# Autodesk Inventor assembly: drivetrain.asm
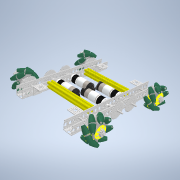
[picture p0: Inventor's stored thumbnail of the model, 180x180]
Saved by Autodesk Inventor 2020 (Build 240168000, 168)
## iProperties
Created: 2019-09-15
Part Number: drivetrain.asm
Document SubType Name: Assembly
Designer: tdmp4
Author: tdmp4
## Documents named in this file (23)
- C:\Users\tdmp4\OneDrive\Documents\GitHub\CAD-2020\Drivetrain\drivetrain.asm.iam
- C:\Users\tdmp4\OneDrive\Documents\GitHub\CAD-2020\ServoCity\585462_cut_17-5.ipt
- C:\Users\tdmp4\OneDrive\Documents\GitHub\CAD-2020\ServoCity\585424.ipt
- C:\Users\tdmp4\OneDrive\Documents\GitHub\CAD-2020\Drivetrain\4_Mecanum_Wheel_276-1447.ipt
- C:\Users\tdmp4\OneDrive\Documents\GitHub\CAD-2020\Drivetrain\GoodAdap.ipt
- C:\Users\tdmp4\OneDrive\Documents\GitHub\CAD-2020\Drivetrain\MirrorGoodAdap.ipt
- C:\Users\tdmp4\OneDrive\Documents\GitHub\CAD-2020\ServoCity\535198.ipt
- C:\Users\tdmp4\OneDrive\Documents\GitHub\CAD-2020\ServoCity\634080.ipt
- C:\Users\tdmp4\OneDrive\Documents\GitHub\CAD-2020\ServoCity\545619 assembly_MIR.ipt
- C:\Users\tdmp4\OneDrive\Documents\GitHub\CAD-2020\ServoCity\615114.ipt
- C:\Users\tdmp4\OneDrive\Documents\GitHub\CAD-2020\ServoCity\555128 assembly.ipt
- C:\Users\tdmp4\OneDrive\Documents\GitHub\CAD-2020\AndyMark\am-3637 NeveRest Orbital 20 Gearmotor REV2.ipt
- C:\Users\tdmp4\OneDrive\Documents\GitHub\CAD-2020\ServoCity\625051 assembly.ipt
- C:\Users\tdmp4\OneDrive\Documents\GitHub\CAD-2020\ServoCity\585462_cut_17-5_MIR.ipt
- C:\Users\tdmp4\OneDrive\Documents\GitHub\CAD-2020\ServoCity\585424_MIR.ipt
- C:\Users\tdmp4\OneDrive\Documents\GitHub\CAD-2020\Drivetrain\4_Mecanum_Wheel_276-1447_MIR.ipt
- C:\Users\tdmp4\OneDrive\Documents\GitHub\CAD-2020\Drivetrain\GoodAdap_MIR.ipt
- C:\Users\tdmp4\OneDrive\Documents\GitHub\CAD-2020\Drivetrain\MirrorGoodAdap_MIR.ipt
- C:\Users\tdmp4\OneDrive\Documents\GitHub\CAD-2020\ServoCity\535198_MIR.ipt
- C:\Users\tdmp4\OneDrive\Documents\GitHub\CAD-2020\ServoCity\634080_MIR.ipt
- C:\Users\tdmp4\OneDrive\Documents\GitHub\CAD-2020\ServoCity\615114_MIR.ipt
- C:\Users\tdmp4\OneDrive\Documents\GitHub\CAD-2020\Drivetrain\1010-Yellow-8_5-CL.ipt
- C:\Users\tdmp4\OneDrive\Documents\GitHub\CAD-2020\ServoCity\634068.ipt
## Components (72 placed, 22 different names)
1. 585462_cut_17-5:1 — Mate:1, Mate:2, Mate:3, Mate:17, Mate:18, Mate:33, Mate:34, Mate:35, Mate:38, Mate:39, Mate:57, Mate:58, Mate:59, Flush:4, Mate:62, Mate:63, Mate:64, Mate:68, Mate:70, Mate:71, Mate:72, Mate:73, Mate:74, Mate:154, Mate:156
2. 585424:1 — Mate:1, Mate:2, Mate:3, Mate:15, Mate:16
3. 4_Mecanum_Wheel_276-1447:1 — Mate:11, Mate:12, Mate:13, Mate:14
4. 4_Mecanum_Wheel_276-1447:2 — Mate:40, Mate:41, Mate:42, Mate:43
5. GoodAdap:1 — Mate:11, Mate:12, Mate:23, Mate:24, Mate:25
6. MirrorGoodAdap:1 — Mate:13, Mate:14, Mate:26, Mate:27, Mate:28, Mate:31
7. 535198:1 — Mate:15, Mate:16, Flush:2
8. 535198:2 — Mate:17, Mate:18, Mate:19
9. 634080:1 — Flush:2, Mate:19, Mate:32
10. 545619 assembly_MIR:1 — Mate:29, Mate:30, Mate:31, Mate:32, Mate:33
11. 545619 assembly_MIR:2 — Mate:23, Mate:24, Mate:25
12. 615114:1 — Mate:26, Mate:27, Mate:28, Mate:29, Mate:30
13. 585424:2 — Mate:34, Mate:35, Mate:36, Mate:37, Flush:4
14. 535198:3 — Mate:36, Mate:37, Mate:54, Flush:3
15. 535198:4 — Mate:38, Mate:39, Mate:56
16. MirrorGoodAdap:2 — Mate:40, Mate:41, Mate:44, Mate:45, Mate:46
17. GoodAdap:2 — Mate:42, Mate:43, Mate:51, Mate:52, Mate:53
18. 615114:2 — Mate:44, Mate:45, Mate:46, Mate:47, Mate:48, Mate:49, Mate:50
19. 545619 assembly_MIR:3 — Mate:47, Mate:48, Mate:49, Mate:50, Mate:55, Mate:56
20. 545619 assembly_MIR:4 — Mate:51, Mate:52, Mate:53
21. 634080:2 — Mate:54, Flush:3, Mate:55
22. 555128 assembly:1 — Mate:57, Mate:58, Mate:59, Mate:60, Mate:61
23. 555128 assembly:2 — Mate:62, Mate:63, Mate:64, Mate:65, Mate:66
24. am-3637 NeveRest Orbital 20 Gearmotor REV2:1 — Mate:60, Mate:61, Mate:69, Mate:163
25. am-3637 NeveRest Orbital 20 Gearmotor REV2:2 — Mate:65, Mate:66, Mate:67, Mate:161
26. 625051 assembly:1 — Mate:67, Mate:68
27. 625051 assembly:2 — Mate:69, Mate:70
28. 535198:5 — Mate:71, Mate:72, Mate:162, Mate:178
29. 535198:6 — Mate:73, Mate:74, Mate:160, Mate:176
30. 585462_cut_17-5_MIR:1 — Mate:75, Mate:76, Mate:77, Mate:84, Mate:85, Mate:87, Flush:6, Mate:98, Mate:99, Mate:102, Mate:103, Mate:144, Mate:145, Mate:146, Mate:147, Mate:148, Mate:149, Flush:11, Mate:164, Mate:165, Mate:166, Mate:167, Mate:175
31. 585424_MIR:1 — Mate:75, Mate:76, Mate:77, Mate:82, Mate:83
32. 4_Mecanum_Wheel_276-1447_MIR:1 — Mate:78, Mate:79, Mate:80, Mate:81
33. 4_Mecanum_Wheel_276-1447_MIR:2 — Mate:104, Mate:105, Mate:106, Mate:107
34. GoodAdap_MIR:1 — Mate:78, Mate:79, Mate:90, Mate:91, Mate:92
35. MirrorGoodAdap_MIR:1 — Mate:80, Mate:81, Mate:89, Mate:95, Mate:96, Mate:97
36. 535198_MIR:1 — Mate:82, Mate:83, Flush:5
37. 535198_MIR:2 — Mate:84, Mate:85, Mate:86
38. 634080_MIR:1 — Mate:86, Flush:5, Mate:88
39. 545619 assembly_MIR:1 — Mate:87, Mate:88, Mate:89, Mate:93, Mate:94
40. 545619 assembly_MIR:2 — Mate:90, Mate:91, Mate:92
41. 615114_MIR:1 — Mate:93, Mate:94, Mate:95, Mate:96, Mate:97
42. 585424_MIR:2 — Flush:6, Mate:98, Mate:99, Mate:100, Mate:101
43. 535198_MIR:3 — Mate:100, Mate:101, Flush:7, Mate:120
44. 535198_MIR:4 — Mate:102, Mate:103, Mate:111
45. MirrorGoodAdap_MIR:2 — Mate:104, Mate:105, Mate:108, Mate:109, Mate:110
46. GoodAdap_MIR:2 — Mate:106, Mate:107, Mate:116, Mate:117, Mate:118
47. 615114_MIR:2 — Mate:108, Mate:109, Mate:110, Mate:112, Mate:113, Mate:114, Mate:115
48. 545619 assembly_MIR:3 — Mate:111, Mate:112, Mate:113, Mate:114, Mate:115, Mate:119
49. 545619 assembly_MIR:4 — Mate:116, Mate:117, Mate:118
50. 634080_MIR:2 — Mate:119, Flush:7, Mate:120
51. 555128 assembly:3 — Mate:144, Mate:145, Mate:146, Mate:150, Mate:151
52. 555128 assembly:4 — Mate:147, Mate:148, Mate:149, Mate:152, Mate:153
53. am-3637 NeveRest Orbital 20 Gearmotor REV2:3 — Mate:150, Mate:151, Mate:159, Flush:14, Mate:169
54. am-3637 NeveRest Orbital 20 Gearmotor REV2:4 — Mate:152, Mate:153, Mate:158, Flush:13, Mate:171
55. 1010-Yellow-8_5-CL:1 — Mate:154, Flush:11
56. 1010-Yellow-8_5-CL:2 — Mate:156
57. 625051 assembly:3 — Mate:159, Flush:14
58. 625051 assembly:5 — Mate:158, Flush:13, Mate:170
59. 634068:1 — Mate:160, Mate:161, Mate:177
60. 634068:2 — Mate:170, Mate:171, Mate:173
61. 634068:3 — Mate:168, Mate:169, Mate:174
62. 634068:4 — Mate:162, Mate:163, Mate:179
63. 535198:7 — Mate:166, Mate:167, Mate:168
64. 535198:8 — Mate:164, Mate:165, Mate:172
65. 545619 assembly_MIR:5 — Mate:172, Mate:173, Mate:189, Mate:190, Mate:191
66. 545619 assembly_MIR:6 — Mate:178, Mate:179, Mate:183, Mate:184, Mate:185
67. 545619 assembly_MIR:7 — Mate:174, Mate:175, Mate:186, Mate:187, Mate:188
68. 545619 assembly_MIR:8 — Mate:176, Mate:177, Mate:180, Mate:181, Mate:182
69. 615114_MIR:3 — Mate:180, Mate:181, Mate:182
70. 615114_MIR:4 — Mate:183, Mate:184, Mate:185
71. 615114_MIR:5 — Mate:186, Mate:187, Mate:188
72. 615114_MIR:6 — Mate:189, Mate:190, Mate:191
## Relationships (165: Mate 156, Flush 9)
- Mate:1: 585462_cut_17-5:1 ↔ 585424:1
- Mate:2 (-38.1 mm): 585462_cut_17-5:1 ↔ 585424:1
- Mate:3: 585462_cut_17-5:1 ↔ 585424:1
- Mate:11: 4_Mecanum_Wheel_276-1447:1 ↔ GoodAdap:1
- Mate:12: 4_Mecanum_Wheel_276-1447:1 ↔ GoodAdap:1
- Mate:13: 4_Mecanum_Wheel_276-1447:1 ↔ MirrorGoodAdap:1
- Mate:14: 4_Mecanum_Wheel_276-1447:1 ↔ MirrorGoodAdap:1
- Mate:15: 585424:1 ↔ 535198:1
- Mate:16: 585424:1 ↔ 535198:1
- Mate:17: 585462_cut_17-5:1 ↔ 535198:2
- Mate:18: 585462_cut_17-5:1 ↔ 535198:2
- Flush:2 (-12.7 mm): 535198:1 ↔ 634080:1
- Mate:19: 535198:2 ↔ 634080:1
- Mate:23: GoodAdap:1 ↔ 545619 assembly_MIR:2
- Mate:24: GoodAdap:1 ↔ 545619 assembly_MIR:2
- Mate:25: GoodAdap:1 ↔ 545619 assembly_MIR:2
- Mate:26 (10.16 mm): MirrorGoodAdap:1 ↔ 615114:1
- Mate:27: MirrorGoodAdap:1 ↔ 615114:1
- Mate:28: MirrorGoodAdap:1 ↔ 615114:1
- Mate:29: 545619 assembly_MIR:1 ↔ 615114:1
- Mate:30: 545619 assembly_MIR:1 ↔ 615114:1
- Mate:31: MirrorGoodAdap:1 ↔ 545619 assembly_MIR:1
- Mate:32: 634080:1 ↔ 545619 assembly_MIR:1
- Mate:33: 585462_cut_17-5:1 ↔ 545619 assembly_MIR:1
- Mate:34: 585462_cut_17-5:1 ↔ 585424:2
- Mate:35: 585462_cut_17-5:1 ↔ 585424:2
- Mate:36: 585424:2 ↔ 535198:3
- Mate:37: 585424:2 ↔ 535198:3
- Mate:38: 585462_cut_17-5:1 ↔ 535198:4
- Mate:39: 585462_cut_17-5:1 ↔ 535198:4
- Mate:40: 4_Mecanum_Wheel_276-1447:2 ↔ MirrorGoodAdap:2
- Mate:41: 4_Mecanum_Wheel_276-1447:2 ↔ MirrorGoodAdap:2
- Mate:42: 4_Mecanum_Wheel_276-1447:2 ↔ GoodAdap:2
- Mate:43: 4_Mecanum_Wheel_276-1447:2 ↔ GoodAdap:2
- Mate:44 (10.16 mm): MirrorGoodAdap:2 ↔ 615114:2
- Mate:45: MirrorGoodAdap:2 ↔ 615114:2
- Mate:46: MirrorGoodAdap:2 ↔ 615114:2
- Mate:47: 615114:2 ↔ 545619 assembly_MIR:3
- Mate:48: 615114:2 ↔ 545619 assembly_MIR:3
- Mate:49: 615114:2 ↔ 545619 assembly_MIR:3
- Mate:50: 615114:2 ↔ 545619 assembly_MIR:3
- Mate:51: GoodAdap:2 ↔ 545619 assembly_MIR:4
- Mate:52: GoodAdap:2 ↔ 545619 assembly_MIR:4
- Mate:53: GoodAdap:2 ↔ 545619 assembly_MIR:4
- Mate:54: 535198:3 ↔ 634080:2
- Flush:3 (-12.7 mm): 535198:3 ↔ 634080:2
- Mate:55: 545619 assembly_MIR:3 ↔ 634080:2
- Mate:56: 535198:4 ↔ 545619 assembly_MIR:3
- Mate:57: 585462_cut_17-5:1 ↔ 555128 assembly:1
- Mate:58: 585462_cut_17-5:1 ↔ 555128 assembly:1
- Mate:59: 585462_cut_17-5:1 ↔ 555128 assembly:1
- Flush:4: 585462_cut_17-5:1 ↔ 585424:2
- Mate:60: 555128 assembly:1 ↔ am-3637 NeveRest Orbital 20 Gearmotor REV2:1
- Mate:61: 555128 assembly:1 ↔ am-3637 NeveRest Orbital 20 Gearmotor REV2:1
- Mate:62: 585462_cut_17-5:1 ↔ 555128 assembly:2
- Mate:63: 585462_cut_17-5:1 ↔ 555128 assembly:2
- Mate:64: 585462_cut_17-5:1 ↔ 555128 assembly:2
- Mate:65: 555128 assembly:2 ↔ am-3637 NeveRest Orbital 20 Gearmotor REV2:2
- Mate:66: 555128 assembly:2 ↔ am-3637 NeveRest Orbital 20 Gearmotor REV2:2
- Mate:67: am-3637 NeveRest Orbital 20 Gearmotor REV2:2 ↔ 625051 assembly:1
- Mate:68 (11.43 mm): 585462_cut_17-5:1 ↔ 625051 assembly:1
- Mate:69: am-3637 NeveRest Orbital 20 Gearmotor REV2:1 ↔ 625051 assembly:2
- Mate:70 (11.43 mm): 585462_cut_17-5:1 ↔ 625051 assembly:2
- Mate:71: 585462_cut_17-5:1 ↔ 535198:5
- Mate:72: 585462_cut_17-5:1 ↔ 535198:5
- Mate:73: 585462_cut_17-5:1 ↔ 535198:6
- Mate:74: 585462_cut_17-5:1 ↔ 535198:6
- Mate:75: 585462_cut_17-5_MIR:1 ↔ 585424_MIR:1
- Mate:76 (-38.1 mm): 585462_cut_17-5_MIR:1 ↔ 585424_MIR:1
- Mate:77: 585462_cut_17-5_MIR:1 ↔ 585424_MIR:1
- Mate:78: 4_Mecanum_Wheel_276-1447_MIR:1 ↔ GoodAdap_MIR:1
- Mate:79: 4_Mecanum_Wheel_276-1447_MIR:1 ↔ GoodAdap_MIR:1
- Mate:80: 4_Mecanum_Wheel_276-1447_MIR:1 ↔ MirrorGoodAdap_MIR:1
- Mate:81: 4_Mecanum_Wheel_276-1447_MIR:1 ↔ MirrorGoodAdap_MIR:1
- Mate:82: 585424_MIR:1 ↔ 535198_MIR:1
- Mate:83: 585424_MIR:1 ↔ 535198_MIR:1
- Mate:84: 585462_cut_17-5_MIR:1 ↔ 535198_MIR:2
- Mate:85: 585462_cut_17-5_MIR:1 ↔ 535198_MIR:2
- Mate:86: 535198_MIR:2 ↔ 634080_MIR:1
- Flush:5 (-12.7 mm): 535198_MIR:1 ↔ 634080_MIR:1
- Mate:87: 585462_cut_17-5_MIR:1 ↔ 545619 assembly_MIR:1
- Mate:88: 634080_MIR:1 ↔ 545619 assembly_MIR:1
- Mate:89: MirrorGoodAdap_MIR:1 ↔ 545619 assembly_MIR:1
- Mate:90: GoodAdap_MIR:1 ↔ 545619 assembly_MIR:2
- Mate:91: GoodAdap_MIR:1 ↔ 545619 assembly_MIR:2
- Mate:92: GoodAdap_MIR:1 ↔ 545619 assembly_MIR:2
- Mate:93: 545619 assembly_MIR:1 ↔ 615114_MIR:1
- Mate:94: 545619 assembly_MIR:1 ↔ 615114_MIR:1
- Mate:95 (10.16 mm): MirrorGoodAdap_MIR:1 ↔ 615114_MIR:1
- Mate:96: MirrorGoodAdap_MIR:1 ↔ 615114_MIR:1
- Mate:97: MirrorGoodAdap_MIR:1 ↔ 615114_MIR:1
- Flush:6: 585462_cut_17-5_MIR:1 ↔ 585424_MIR:2
- Mate:98: 585462_cut_17-5_MIR:1 ↔ 585424_MIR:2
- Mate:99: 585462_cut_17-5_MIR:1 ↔ 585424_MIR:2
- Mate:100: 585424_MIR:2 ↔ 535198_MIR:3
- Mate:101: 585424_MIR:2 ↔ 535198_MIR:3
- Mate:102: 585462_cut_17-5_MIR:1 ↔ 535198_MIR:4
- Mate:103: 585462_cut_17-5_MIR:1 ↔ 535198_MIR:4
- Mate:104: 4_Mecanum_Wheel_276-1447_MIR:2 ↔ MirrorGoodAdap_MIR:2
- Mate:105: 4_Mecanum_Wheel_276-1447_MIR:2 ↔ MirrorGoodAdap_MIR:2
- Mate:106: 4_Mecanum_Wheel_276-1447_MIR:2 ↔ GoodAdap_MIR:2
- Mate:107: 4_Mecanum_Wheel_276-1447_MIR:2 ↔ GoodAdap_MIR:2
- Mate:108: MirrorGoodAdap_MIR:2 ↔ 615114_MIR:2
- Mate:109: MirrorGoodAdap_MIR:2 ↔ 615114_MIR:2
- Mate:110 (10.16 mm): MirrorGoodAdap_MIR:2 ↔ 615114_MIR:2
- Mate:111: 535198_MIR:4 ↔ 545619 assembly_MIR:3
- Mate:112: 615114_MIR:2 ↔ 545619 assembly_MIR:3
- Mate:113: 615114_MIR:2 ↔ 545619 assembly_MIR:3
- Mate:114: 615114_MIR:2 ↔ 545619 assembly_MIR:3
- Mate:115: 615114_MIR:2 ↔ 545619 assembly_MIR:3
- Mate:116: GoodAdap_MIR:2 ↔ 545619 assembly_MIR:4
- Mate:117: GoodAdap_MIR:2 ↔ 545619 assembly_MIR:4
- Mate:118: GoodAdap_MIR:2 ↔ 545619 assembly_MIR:4
- Mate:119: 545619 assembly_MIR:3 ↔ 634080_MIR:2
- Flush:7 (-12.7 mm): 535198_MIR:3 ↔ 634080_MIR:2
- Mate:120: 535198_MIR:3 ↔ 634080_MIR:2
- Mate:144: 585462_cut_17-5_MIR:1 ↔ 555128 assembly:3
- Mate:145: 585462_cut_17-5_MIR:1 ↔ 555128 assembly:3
- Mate:146: 585462_cut_17-5_MIR:1 ↔ 555128 assembly:3
- Mate:147: 585462_cut_17-5_MIR:1 ↔ 555128 assembly:4
- Mate:148: 585462_cut_17-5_MIR:1 ↔ 555128 assembly:4
- Mate:149: 585462_cut_17-5_MIR:1 ↔ 555128 assembly:4
- Mate:150: 555128 assembly:3 ↔ am-3637 NeveRest Orbital 20 Gearmotor REV2:3
- Mate:151: 555128 assembly:3 ↔ am-3637 NeveRest Orbital 20 Gearmotor REV2:3
- Mate:152: 555128 assembly:4 ↔ am-3637 NeveRest Orbital 20 Gearmotor REV2:4
- Mate:153: 555128 assembly:4 ↔ am-3637 NeveRest Orbital 20 Gearmotor REV2:4
- Mate:154: 585462_cut_17-5:1 ↔ 1010-Yellow-8_5-CL:1
- Flush:11 (107.95 mm): 585462_cut_17-5_MIR:1 ↔ 1010-Yellow-8_5-CL:1
- Mate:156: 585462_cut_17-5:1 ↔ 1010-Yellow-8_5-CL:2
- Mate:158: am-3637 NeveRest Orbital 20 Gearmotor REV2:4 ↔ 625051 assembly:5
- Flush:13 (-5.08 mm): am-3637 NeveRest Orbital 20 Gearmotor REV2:4 ↔ 625051 assembly:5
- Mate:159: am-3637 NeveRest Orbital 20 Gearmotor REV2:3 ↔ 625051 assembly:3
- Flush:14 (-5.08 mm): am-3637 NeveRest Orbital 20 Gearmotor REV2:3 ↔ 625051 assembly:3
- Mate:160: 535198:6 ↔ 634068:1
- Mate:161: am-3637 NeveRest Orbital 20 Gearmotor REV2:2 ↔ 634068:1
- Mate:162: 535198:5 ↔ 634068:4
- Mate:163: am-3637 NeveRest Orbital 20 Gearmotor REV2:1 ↔ 634068:4
- Mate:164: 585462_cut_17-5_MIR:1 ↔ 535198:8
- Mate:165: 585462_cut_17-5_MIR:1 ↔ 535198:8
- Mate:166: 585462_cut_17-5_MIR:1 ↔ 535198:7
- Mate:167: 585462_cut_17-5_MIR:1 ↔ 535198:7
- Mate:168: 634068:3 ↔ 535198:7
- Mate:169: am-3637 NeveRest Orbital 20 Gearmotor REV2:3 ↔ 634068:3
- Mate:170: 625051 assembly:5 ↔ 634068:2
- Mate:171: am-3637 NeveRest Orbital 20 Gearmotor REV2:4 ↔ 634068:2
- Mate:172: 535198:8 ↔ 545619 assembly_MIR:5
- Mate:173: 634068:2 ↔ 545619 assembly_MIR:5
- Mate:174: 634068:3 ↔ 545619 assembly_MIR:7
- Mate:175: 585462_cut_17-5_MIR:1 ↔ 545619 assembly_MIR:7
- Mate:176: 535198:6 ↔ 545619 assembly_MIR:8
- Mate:177: 634068:1 ↔ 545619 assembly_MIR:8
- Mate:178: 535198:5 ↔ 545619 assembly_MIR:6
- Mate:179: 634068:4 ↔ 545619 assembly_MIR:6
- Mate:180: 545619 assembly_MIR:8 ↔ 615114_MIR:3
- Mate:181: 545619 assembly_MIR:8 ↔ 615114_MIR:3
- Mate:182: 545619 assembly_MIR:8 ↔ 615114_MIR:3
- Mate:183: 545619 assembly_MIR:6 ↔ 615114_MIR:4
- Mate:184: 545619 assembly_MIR:6 ↔ 615114_MIR:4
- Mate:185: 545619 assembly_MIR:6 ↔ 615114_MIR:4
- Mate:186: 545619 assembly_MIR:7 ↔ 615114_MIR:5
- Mate:187: 545619 assembly_MIR:7 ↔ 615114_MIR:5
- Mate:188: 545619 assembly_MIR:7 ↔ 615114_MIR:5
- Mate:189: 545619 assembly_MIR:5 ↔ 615114_MIR:6
- Mate:190: 545619 assembly_MIR:5 ↔ 615114_MIR:6
- Mate:191: 545619 assembly_MIR:5 ↔ 615114_MIR:6
